# Autodesk Inventor assembly: HeildarAssembly
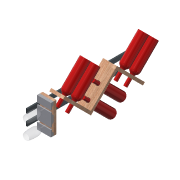
[picture p0: Inventor's stored thumbnail of the model, 180x180]
Saved by Autodesk Inventor 2018 (Build 220112000, 112)
## iProperties
Created: 2020-03-01
Part Number: HeildarAssembly
Document SubType Name: Assembly
Designer: Spark
Author: Spark
## Documents named in this file (8)
- C:\Users\ottar\OneDrive\Skjáborð\Skoli\6. misseri\Framleiðsluferli\Verkefni 4 - Lokaverkefni\HeildarAssembly.iam
- C:\Users\ottar\OneDrive\Skjáborð\Skoli\6. misseri\Framleiðsluferli\Verkefni 4 - Lokaverkefni\EndaHaldarar.ipt
- C:\Users\ottar\OneDrive\Skjáborð\Skoli\6. misseri\Framleiðsluferli\Verkefni 4 - Lokaverkefni\MidjuHaldarar.ipt
- C:\Users\ottar\OneDrive\Skjáborð\Skoli\6. misseri\Framleiðsluferli\Verkefni 4 - Lokaverkefni\WINE_RED_1.ipt
- C:\Users\ottar\OneDrive\Skjáborð\Skoli\6. misseri\Framleiðsluferli\Verkefni 4 - Lokaverkefni\BackPlates.ipt
- C:\Users\ottar\OneDrive\Skjáborð\Skoli\6. misseri\Framleiðsluferli\Verkefni 4 - Lokaverkefni\GlassHolder.ipt
- C:\Users\ottar\OneDrive\Skjáborð\Skoli\6. misseri\Framleiðsluferli\Verkefni 4 - Lokaverkefni\Vínglasahaldari-v4.iam
- C:\Users\ottar\OneDrive\Skjáborð\Skoli\6. misseri\Framleiðsluferli\Verkefni 4 - Lokaverkefni\RED WINE GLASS.ipt
## Components (18 placed, 7 different names)
1. EndaHaldarar:1 — Flush:11, Flush:21, Flush:22, Mate:30, Mate:31, Flush:23, Flush:24
2. MidjuHaldarar:1 — Mate:12, Mate:13, Flush:11, Flush:12, Mate:20, Mate:25, Mate:26, Flush:16, Flush:17, Flush:20, Mate:29, Flush:21, Flush:22
3. EndaHaldarar:2 — Flush:12, Mate:23, Flush:14, Flush:15, Mate:24, Flush:20, Mate:29
4. BackPlates:1 — Mate:12, Mate:14, Flush:9, Mate:20, Mate:21, Mate:22
5. BackPlates:2 — Mate:13, Mate:14, Flush:9, Mate:15
6. GlassHolder:1 — Mate:22, Flush:25, Flush:27, Mate:36, Flush:29, Mate:37, Flush:30, Mate:39, Flush:33, Mate:41, Mate:43, Mate:44, Mate:46
7. WINE_RED_1:1 — Flush:15, Mate:24
8. WINE_RED_1:2 — Mate:26, Flush:16
9. WINE_RED_1:3 — Mate:31, Flush:23
10. WINE_RED_1:4 — Mate:30, Flush:24
11. WINE_RED_1:5 — Mate:23, Flush:14
12. WINE_RED_1:6 — Mate:25, Flush:17
13. Vínglasahaldari-v4:1 [sub-assembly] — Flush:25, Mate:36, Flush:29, Mate:40, Mate:42
14. Vínglasahaldari-v4:2 [sub-assembly] — Flush:27, Mate:37, Flush:30
15. Vínglasahaldari-v4:3 [sub-assembly] — Mate:38, Flush:31, Flush:32, Mate:45
16. Vínglasahaldari-v4:4 [sub-assembly] — Mate:38, Flush:31, Flush:32, Mate:39, Flush:33, Mate:40
17. RED WINE GLASS:1 — Mate:44, Mate:45, Mate:46
18. RED WINE GLASS:2 — Mate:41, Mate:42, Mate:43
## Relationships (44: Mate 25, Flush 19)
- Mate:12: MidjuHaldarar:1 ↔ BackPlates:1
- Mate:13: MidjuHaldarar:1 ↔ BackPlates:2
- Mate:14 (50 mm): BackPlates:1 ↔ BackPlates:2
- Flush:9: BackPlates:1 ↔ BackPlates:2
- Mate:15: BackPlates:2
- Flush:11: EndaHaldarar:1 ↔ MidjuHaldarar:1
- Flush:12: MidjuHaldarar:1 ↔ EndaHaldarar:2
- Mate:20 (25 mm): MidjuHaldarar:1 ↔ BackPlates:1
- Mate:21: BackPlates:1
- Mate:22: BackPlates:1 ↔ GlassHolder:1
- Mate:23: EndaHaldarar:2 ↔ WINE_RED_1:5
- Flush:14 (-50 mm): EndaHaldarar:2 ↔ WINE_RED_1:5
- Flush:15 (-50 mm): EndaHaldarar:2 ↔ WINE_RED_1:1
- Mate:24: EndaHaldarar:2 ↔ WINE_RED_1:1
- Mate:25: MidjuHaldarar:1 ↔ WINE_RED_1:6
- Mate:26: MidjuHaldarar:1 ↔ WINE_RED_1:2
- Flush:16 (-50 mm): MidjuHaldarar:1 ↔ WINE_RED_1:2
- Flush:17 (50 mm): MidjuHaldarar:1 ↔ WINE_RED_1:6
- Flush:20: MidjuHaldarar:1 ↔ EndaHaldarar:2
- Mate:29: MidjuHaldarar:1 ↔ EndaHaldarar:2
- Flush:21: EndaHaldarar:1 ↔ MidjuHaldarar:1
- Flush:22: EndaHaldarar:1 ↔ MidjuHaldarar:1
- Mate:30: EndaHaldarar:1 ↔ WINE_RED_1:4
- Mate:31: EndaHaldarar:1 ↔ WINE_RED_1:3
- Flush:23 (-50 mm): EndaHaldarar:1 ↔ WINE_RED_1:3
- Flush:24 (50 mm): EndaHaldarar:1 ↔ WINE_RED_1:4
- Flush:25: GlassHolder:1 ↔ Vínglasahaldari-v4:1
- Flush:27: GlassHolder:1 ↔ Vínglasahaldari-v4:2
- Mate:36: GlassHolder:1 ↔ Vínglasahaldari-v4:1
- Flush:29: GlassHolder:1 ↔ Vínglasahaldari-v4:1
- Mate:37: GlassHolder:1 ↔ Vínglasahaldari-v4:2
- Flush:30: GlassHolder:1 ↔ Vínglasahaldari-v4:2
- Mate:38: Vínglasahaldari-v4:3 ↔ Vínglasahaldari-v4:4
- Flush:31: Vínglasahaldari-v4:3 ↔ Vínglasahaldari-v4:4
- Flush:32: Vínglasahaldari-v4:3 ↔ Vínglasahaldari-v4:4
- Mate:39: GlassHolder:1 ↔ Vínglasahaldari-v4:4
- Flush:33: GlassHolder:1 ↔ Vínglasahaldari-v4:4
- Mate:40 (14.834 mm): Vínglasahaldari-v4:1 ↔ Vínglasahaldari-v4:4
- Mate:41 (5 mm): GlassHolder:1 ↔ RED WINE GLASS:2
- Mate:42 (7 mm): Vínglasahaldari-v4:1 ↔ RED WINE GLASS:2
- Mate:43 (-40 mm): GlassHolder:1 ↔ RED WINE GLASS:2
- Mate:44 (5 mm): GlassHolder:1 ↔ RED WINE GLASS:1
- Mate:45 (7 mm): Vínglasahaldari-v4:3 ↔ RED WINE GLASS:1
- Mate:46 (-40 mm): GlassHolder:1 ↔ RED WINE GLASS:1
